# Autodesk Inventor assembly: Assembly1
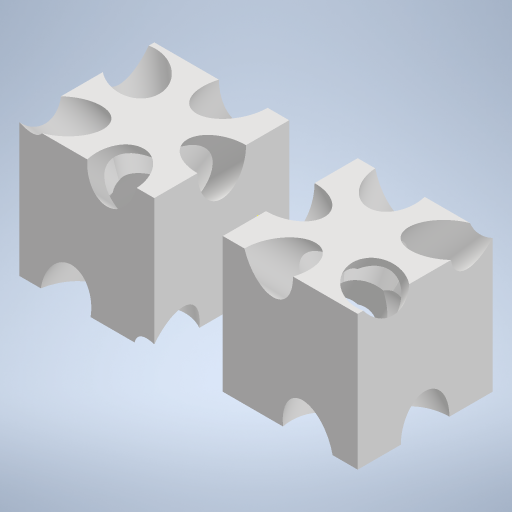
[picture p0: Inventor's stored thumbnail of the model, 512x512]
Saved by Autodesk Inventor 2024 (Build 280153020, 153B)
## iProperties
Created: 2023-11-21
Part Number: Assembly1
Document SubType Name: Assembly
Designer: 5802269
Author: 5802269
## Documents named in this file (2)
- M:\CS 30\Assembly1.iam
- M:\CS 30\Part1.ipt
## Components (2 placed, 1 different names)
1. Part1:1 — Mate:1, Flush:1
2. Part1:2 — Mate:1, Flush:1
## Relationships (2: Mate 1, Flush 1)
- Mate:1 (12.7 mm): Part1:1 ↔ Part1:2
- Flush:1: Part1:1 ↔ Part1:2
